# Autodesk Inventor assembly: Chasis
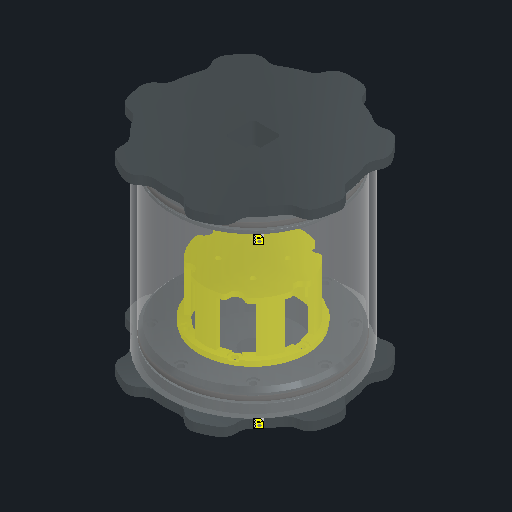
[picture p0: Inventor's stored thumbnail of the model, 512x512]
Saved by Autodesk Inventor 2025.4 (Build 294407000, 407)
## iProperties
Created: 2025-10-11
Part Number: Chasis
Document SubType Name: Assembly
Designer: santa
Author: santa
## Documents named in this file (7)
- C:\Users\danie\OneDrive\Documentos\Inventor\Arbol\V4\V4\Chasis.iam
- C:\Users\danie\OneDrive\Documentos\Inventor\Arbol\V4\V4\Chasis\Tapa_Inferior.ipt
- C:\Users\danie\OneDrive\Documentos\Inventor\Arbol\V4\V4\Chasis\Tapa_Superior.ipt
- C:\Users\danie\OneDrive\Documentos\Inventor\Arbol\V4\V4\Chasis\Tuberia.ipt
- C:\Users\danie\OneDrive\Documentos\Inventor\Arbol\V4\V4\O'Ring\1.78.ipt
- C:\Users\danie\OneDrive\Documentos\Inventor\Arbol\V4\V4\O'Ring\2.62.ipt
- C:\Users\danie\OneDrive\Documentos\Inventor\Arbol\V4\V4\Chasis\Soporte_Motor.ipt
## Components (8 placed, 6 different names)
1. Tapa_Inferior:1 — Rigid:1, Rigid:3
2. Tuberia:1 — Rigid:1, Rigid:8
3. 1.78:1 — Rigid:10
4. 2.62:1 — Rigid:3
5. 2.62:2 — Rigid:11
6. Soporte_Motor:1 — Rigid:13, Rigid:14
7. 1.78:2 — Rigid:9
8. Tapa_Superior:1 — Rigid:8, Rigid:9, Rigid:10, Rigid:11, Rigid:13, Rigid:14
## Relationships (8: WeldJoint 8)
- Rigid:1 [WeldJoint]: Tapa_Inferior:1 ↔ Tuberia:1
- Rigid:3 [WeldJoint]: Tapa_Inferior:1 ↔ 2.62:1
- Rigid:8 [WeldJoint]: Tuberia:1 ↔ Tapa_Superior:1
- Rigid:9 [WeldJoint] (0.89 mm): 1.78:2 ↔ Tapa_Superior:1
- Rigid:10 [WeldJoint] (0.89 mm): 1.78:1 ↔ Tapa_Superior:1
- Rigid:11 [WeldJoint]: 2.62:2 ↔ Tapa_Superior:1
- Rigid:13 [WeldJoint]: Soporte_Motor:1 ↔ Tapa_Superior:1
- Rigid:14 [WeldJoint]: Soporte_Motor:1 ↔ Tapa_Superior:1
